# Autodesk Inventor assembly: Weapon Assembly
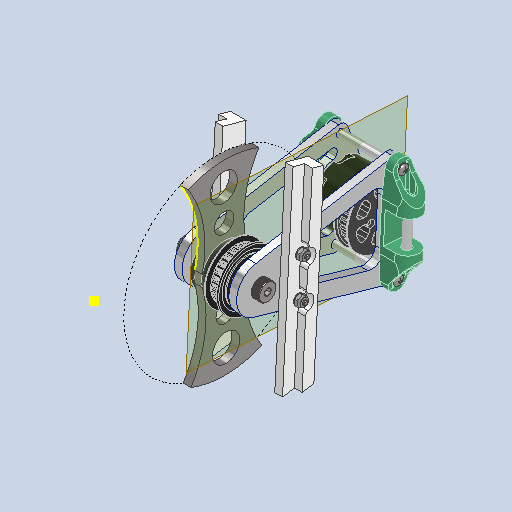
[picture p0: Inventor's stored thumbnail of the model, 512x512]
Saved by Autodesk Inventor 2023.1 (Build 271208000, 208)
## iProperties
Created: 2022-05-21
Part Number: Weapon Assembly
Document SubType Name: Assembly
Designer: Nathan Cai
Mass: 747.016 g
Surface Area: 1345.14 cm^2
Volume: 239.025 cm^3
Density: 3.12526 g/cm^3
Author: Nathan Cai
## Documents named in this file (15)
- C:\Users\Nathan Cai\Documents\Inventor\0.3rd Lawette - V3.5\Vertical Weapon Assembly (Type A - Low Power)\Weapon Assembly (Vert A - Low Power).iam
- C:\Users\Nathan Cai\Documents\Inventor\0.3rd Lawette - V3.5\Vertical Weapon Assembly (Type A)\90807A139_Same-Size Thread Alloy Steel Shoulder Screw.ipt
- C:\Users\Nathan Cai\Documents\Inventor\0.3rd Lawette - V3.5\Vertical Weapon Assembly (Type A)\90630A121_High-Strength Steel Nylon-Insert Locknut.ipt
- C:\Users\Nathan Cai\Documents\Inventor\0.3rd Lawette - V3.5\Vertical Weapon Assembly (Type A)\Frame (Clear Side).ipt
- C:\Users\Nathan Cai\Documents\Inventor\0.3rd Lawette - V3.5\Standoff 1.5in.ipt
- C:\Users\Nathan Cai\Documents\Inventor\0.3rd Lawette - V3.5\Vertical Weapon Assembly (Type A)\Legs.ipt
- C:\Users\Nathan Cai\Documents\Inventor\Content Center Files\R2023\en-US\ANSI B18.6.3(27)\ANSI B18.6.3 - 6-32 UNC - 0.75(11).ipt
- C:\Users\Nathan Cai\Documents\Inventor\Content Center Files\R2023\en-US\SAE J773b\SAE J773b - No. 6. SAE Type L. narrow.ipt
- C:\Users\Nathan Cai\Documents\Inventor\Content Center Files\R2023\en-US\IFI 100 107(2)\IFI 100_107 - No. 6 - 32 Metal Type.ipt
- C:\Users\Nathan Cai\Documents\Inventor\0.3rd Lawette - V3.5\Vertical Weapon Assembly (Type A)\Frame (Motor Side).ipt
- C:\Users\Nathan Cai\Documents\Inventor\0.3rd Lawette - V3.5\Vertical Weapon Assembly (Type A)\Legs_MIR.ipt
- C:\Users\Nathan Cai\Documents\Inventor\0.3rd Lawette - V3.5\Bracket.ipt
- C:\Users\Nathan Cai\Documents\Inventor\Content Center Files\R2023\en-US\ANSI B18.6.3(27)\ANSI B18.6.3 - 6-32 UNC - 0.625(11).ipt
- C:\Users\Nathan Cai\Documents\Inventor\0.3rd Lawette - V3.5\Vertical Weapon Assembly (Type A - Low Power)\Weapon (Weapon-Side Pulley).iam
- C:\Users\Nathan Cai\Documents\Inventor\0.3rd Lawette - V3.5\Vertical Weapon Assembly (Type A - Low Power)\Weapon (Motor-Side Pulley).iam
## Components (42 placed, 14 different names)
1. Weapon (Weapon-Side Pulley):2 [sub-assembly]
2. Weapon (Motor-Side Pulley):2 [sub-assembly]
3. 90807A139_Same-Size Thread Alloy Steel Shoulder Screw:1 — Mate:1, Mate:2, Mate:9, Mate:10
4. 90630A121_High-Strength Steel Nylon-Insert Locknut:1 — Mate:1, Mate:2
5. Frame (Motor Side):1 — Symmetry:1, Mate:146, Mate:147, Mate:148, Mate:170, Mate:194, Mate:195, Mate:196, Mate:197, Mate:198, Mate:200
6. Frame (Clear Side):1 — Mate:9, Mate:10, Mate:28, Mate:29, Mate:30, Mate:102, Symmetry:1, Mate:173, Mate:202, Mate:203, Mate:204, Mate:205, Mate:206, Mate:208
7. Legs:1 — Mate:28, Mate:29, Mate:30, Mate:207, Mate:209
8. Legs_MIR:1 — Mate:146, Mate:147, Mate:148, Mate:199, Mate:201
9. Bracket:1 — Mate:173, Mate:174, Mate:175, Mate:176, Flush:2, Mate:210, Mate:211, Mate:212, Mate:213, Mate:218, Mate:219, Mate:221, Mate:222
10. Bracket:2 — Mate:170, Mate:171, Mate:172, Mate:177, Flush:1, Mate:214, Mate:215, Mate:216, Mate:217, Mate:220, Mate:224
11. Standoff 1.5in:1 — Mate:102, Mate:171, Mate:174
12. Standoff 1.5in:2 — Mate:172, Mate:175
13. Standoff 1.5in:3 — Mate:176, Flush:2, Mate:223, Mate:225
14. Standoff 1.5in:4 — Mate:177, Flush:1
15. Cross Recessed Truss Head Machine Screw - Type I - Inch No. 6 - 32 - 5/8:8 — Insert:44
16. Conical Spring Washer SAE J773b (Inch) No. 6. SAE Type L. narrow:38 — Mate:224, Mate:225, Insert:44
17. Cross Recessed Truss Head Machine Screw - Type I - Inch No. 6 - 32 - 5/8:7 — Insert:43
18. Conical Spring Washer SAE J773b (Inch) No. 6. SAE Type L. narrow:37 — Mate:222, Mate:223, Insert:43
19. Cross Recessed Truss Head Machine Screw - Type I - Inch No. 6 - 32 - 5/8:6 — Insert:42
20. Conical Spring Washer SAE J773b (Inch) No. 6. SAE Type L. narrow:36 — Mate:220, Mate:221, Insert:42
21. Cross Recessed Truss Head Machine Screw - Type I - Inch No. 6 - 32 - 5/8:5 — Insert:41
22. Conical Spring Washer SAE J773b (Inch) No. 6. SAE Type L. narrow:35 — Mate:218, Mate:219, Insert:41
23. Cross Recessed Truss Head Machine Screw - Type I - Inch No. 6 - 32 - 3/4:27 — Insert:40
24. Conical Spring Washer SAE J773b (Inch) No. 6. SAE Type L. narrow:34 — Mate:216, Mate:217, Insert:40
25. Cross Recessed Truss Head Machine Screw - Type I - Inch No. 6 - 32 - 3/4:26 — Insert:39
26. Conical Spring Washer SAE J773b (Inch) No. 6. SAE Type L. narrow:33 — Mate:214, Mate:215, Insert:39
27. Cross Recessed Truss Head Machine Screw - Type I - Inch No. 6 - 32 - 3/4:25 — Insert:38
28. Conical Spring Washer SAE J773b (Inch) No. 6. SAE Type L. narrow:32 — Mate:212, Mate:213, Insert:38
29. Cross Recessed Truss Head Machine Screw - Type I - Inch No. 6 - 32 - 3/4:24 — Insert:37
30. Conical Spring Washer SAE J773b (Inch) No. 6. SAE Type L. narrow:31 — Mate:210, Mate:211, Insert:37
31. Prevailing Torque Type Hex Nut - Inch (IFI) No. 6 - 32 Metal Type:22 — Insert:36
32. Conical Spring Washer SAE J773b (Inch) No. 6. SAE Type L. narrow:30 — Mate:208, Mate:209, Insert:36
33. Cross Recessed Truss Head Machine Screw - Type I - Inch No. 6 - 32 - 3/4:23 — Mate:204, Mate:205
34. Prevailing Torque Type Hex Nut - Inch (IFI) No. 6 - 32 Metal Type:21 — Insert:35
35. Conical Spring Washer SAE J773b (Inch) No. 6. SAE Type L. narrow:29 — Mate:206, Mate:207, Insert:35
36. Cross Recessed Truss Head Machine Screw - Type I - Inch No. 6 - 32 - 3/4:22 — Mate:202, Mate:203
37. Prevailing Torque Type Hex Nut - Inch (IFI) No. 6 - 32 Metal Type:20 — Insert:34
38. Conical Spring Washer SAE J773b (Inch) No. 6. SAE Type L. narrow:28 — Mate:200, Mate:201, Insert:34
39. Cross Recessed Truss Head Machine Screw - Type I - Inch No. 6 - 32 - 3/4:21 — Mate:196, Mate:197
40. Prevailing Torque Type Hex Nut - Inch (IFI) No. 6 - 32 Metal Type:19 — Insert:33
41. Conical Spring Washer SAE J773b (Inch) No. 6. SAE Type L. narrow:27 — Mate:198, Mate:199, Insert:33
42. Cross Recessed Truss Head Machine Screw - Type I - Inch No. 6 - 32 - 3/4:20 — Mate:194, Mate:195
## Relationships (77: Mate 62, Insert 12, Flush 2, Symmetry 1)
- Mate:1: 90807A139_Same-Size Thread Alloy Steel Shoulder Screw:1 ↔ 90630A121_High-Strength Steel Nylon-Insert Locknut:1
- Mate:2 (50.8 mm): 90807A139_Same-Size Thread Alloy Steel Shoulder Screw:1 ↔ 90630A121_High-Strength Steel Nylon-Insert Locknut:1
- [Mate]: Weapon (Weapon-Side Pulley):2 ↔ 90807A139_Same-Size Thread Alloy Steel Shoulder Screw:1
- [Mate]: 90807A139_Same-Size Thread Alloy Steel Shoulder Screw:1 ↔ Frame (Motor Side):1
- Mate:9: 90807A139_Same-Size Thread Alloy Steel Shoulder Screw:1 ↔ Frame (Clear Side):1
- Mate:10: 90807A139_Same-Size Thread Alloy Steel Shoulder Screw:1 ↔ Frame (Clear Side):1
- [Mate]: Frame (Motor Side):1 ↔ Frame (Clear Side):1
- [Mate]: Frame (Motor Side):1 ↔ Standoff 1.5in:1
- [Mate]: Frame (Motor Side):1 ↔ Standoff 1.5in:2
- [Mate]: Frame (Motor Side):1 ↔ Standoff 1.5in:1
- [Mate]: Frame (Motor Side):1 ↔ Standoff 1.5in:2
- Mate:28: Frame (Clear Side):1 ↔ Legs:1
- Mate:29: Frame (Clear Side):1 ↔ Legs:1
- Mate:30: Frame (Clear Side):1 ↔ Legs:1
- Mate:102: Frame (Clear Side):1 ↔ Standoff 1.5in:1
- [Mate] (0.0254 mm): Weapon (Weapon-Side Pulley):2 ↔ Frame (Motor Side):1
- Symmetry:1: Frame (Motor Side):1 ↔ Frame (Clear Side):1
- Mate:146: Frame (Motor Side):1 ↔ Legs_MIR:1
- Mate:147: Frame (Motor Side):1 ↔ Legs_MIR:1
- Mate:148: Frame (Motor Side):1 ↔ Legs_MIR:1
- [Mate]: Weapon (Motor-Side Pulley):2 ↔ Frame (Motor Side):1
- [Mate]: Weapon (Motor-Side Pulley):2 ↔ Frame (Motor Side):1
- [Mate]: Weapon (Motor-Side Pulley):2 ↔ Frame (Motor Side):1
- Mate:170: Frame (Motor Side):1 ↔ Bracket:2
- Mate:171: Bracket:2 ↔ Standoff 1.5in:1
- Mate:172: Bracket:2 ↔ Standoff 1.5in:2
- Mate:173: Frame (Clear Side):1 ↔ Bracket:1
- Mate:174: Bracket:1 ↔ Standoff 1.5in:1
- Mate:175: Bracket:1 ↔ Standoff 1.5in:2
- Mate:176: Bracket:1 ↔ Standoff 1.5in:3
- Mate:177: Bracket:2 ↔ Standoff 1.5in:4
- Flush:1: Bracket:2 ↔ Standoff 1.5in:4
- Flush:2: Bracket:1 ↔ Standoff 1.5in:3
- Mate:194: Frame (Motor Side):1 ↔ Cross Recessed Truss Head Machine Screw - Type I - Inch No. 6 - 32 - 3/4:20
- Mate:195: Frame (Motor Side):1 ↔ Cross Recessed Truss Head Machine Screw - Type I - Inch No. 6 - 32 - 3/4:20
- Mate:196: Frame (Motor Side):1 ↔ Cross Recessed Truss Head Machine Screw - Type I - Inch No. 6 - 32 - 3/4:21
- Mate:197: Frame (Motor Side):1 ↔ Cross Recessed Truss Head Machine Screw - Type I - Inch No. 6 - 32 - 3/4:21
- Mate:198: Frame (Motor Side):1 ↔ Conical Spring Washer SAE J773b (Inch) No. 6. SAE Type L. narrow:27
- Mate:199: Legs_MIR:1 ↔ Conical Spring Washer SAE J773b (Inch) No. 6. SAE Type L. narrow:27
- Mate:200: Frame (Motor Side):1 ↔ Conical Spring Washer SAE J773b (Inch) No. 6. SAE Type L. narrow:28
- Mate:201: Legs_MIR:1 ↔ Conical Spring Washer SAE J773b (Inch) No. 6. SAE Type L. narrow:28
- Insert:33: Prevailing Torque Type Hex Nut - Inch (IFI) No. 6 - 32 Metal Type:19 ↔ Conical Spring Washer SAE J773b (Inch) No. 6. SAE Type L. narrow:27
- Insert:34: Prevailing Torque Type Hex Nut - Inch (IFI) No. 6 - 32 Metal Type:20 ↔ Conical Spring Washer SAE J773b (Inch) No. 6. SAE Type L. narrow:28
- Mate:202: Frame (Clear Side):1 ↔ Cross Recessed Truss Head Machine Screw - Type I - Inch No. 6 - 32 - 3/4:22
- Mate:203: Frame (Clear Side):1 ↔ Cross Recessed Truss Head Machine Screw - Type I - Inch No. 6 - 32 - 3/4:22
- Mate:204: Frame (Clear Side):1 ↔ Cross Recessed Truss Head Machine Screw - Type I - Inch No. 6 - 32 - 3/4:23
- Mate:205: Frame (Clear Side):1 ↔ Cross Recessed Truss Head Machine Screw - Type I - Inch No. 6 - 32 - 3/4:23
- Mate:206: Frame (Clear Side):1 ↔ Conical Spring Washer SAE J773b (Inch) No. 6. SAE Type L. narrow:29
- Mate:207: Legs:1 ↔ Conical Spring Washer SAE J773b (Inch) No. 6. SAE Type L. narrow:29
- Mate:208: Frame (Clear Side):1 ↔ Conical Spring Washer SAE J773b (Inch) No. 6. SAE Type L. narrow:30
- Mate:209: Legs:1 ↔ Conical Spring Washer SAE J773b (Inch) No. 6. SAE Type L. narrow:30
- Insert:35: Prevailing Torque Type Hex Nut - Inch (IFI) No. 6 - 32 Metal Type:21 ↔ Conical Spring Washer SAE J773b (Inch) No. 6. SAE Type L. narrow:29
- Insert:36: Prevailing Torque Type Hex Nut - Inch (IFI) No. 6 - 32 Metal Type:22 ↔ Conical Spring Washer SAE J773b (Inch) No. 6. SAE Type L. narrow:30
- Mate:210: Bracket:1 ↔ Conical Spring Washer SAE J773b (Inch) No. 6. SAE Type L. narrow:31
- Mate:211: Bracket:1 ↔ Conical Spring Washer SAE J773b (Inch) No. 6. SAE Type L. narrow:31
- Mate:212: Bracket:1 ↔ Conical Spring Washer SAE J773b (Inch) No. 6. SAE Type L. narrow:32
- Mate:213: Bracket:1 ↔ Conical Spring Washer SAE J773b (Inch) No. 6. SAE Type L. narrow:32
- Insert:37: Cross Recessed Truss Head Machine Screw - Type I - Inch No. 6 - 32 - 3/4:24 ↔ Conical Spring Washer SAE J773b (Inch) No. 6. SAE Type L. narrow:31
- Insert:38: Cross Recessed Truss Head Machine Screw - Type I - Inch No. 6 - 32 - 3/4:25 ↔ Conical Spring Washer SAE J773b (Inch) No. 6. SAE Type L. narrow:32
- Mate:214: Bracket:2 ↔ Conical Spring Washer SAE J773b (Inch) No. 6. SAE Type L. narrow:33
- Mate:215: Bracket:2 ↔ Conical Spring Washer SAE J773b (Inch) No. 6. SAE Type L. narrow:33
- Mate:216: Bracket:2 ↔ Conical Spring Washer SAE J773b (Inch) No. 6. SAE Type L. narrow:34
- Mate:217: Bracket:2 ↔ Conical Spring Washer SAE J773b (Inch) No. 6. SAE Type L. narrow:34
- Insert:39: Cross Recessed Truss Head Machine Screw - Type I - Inch No. 6 - 32 - 3/4:26 ↔ Conical Spring Washer SAE J773b (Inch) No. 6. SAE Type L. narrow:33
- Insert:40: Cross Recessed Truss Head Machine Screw - Type I - Inch No. 6 - 32 - 3/4:27 ↔ Conical Spring Washer SAE J773b (Inch) No. 6. SAE Type L. narrow:34
- Mate:218: Bracket:1 ↔ Conical Spring Washer SAE J773b (Inch) No. 6. SAE Type L. narrow:35
- Mate:219: Bracket:1 ↔ Conical Spring Washer SAE J773b (Inch) No. 6. SAE Type L. narrow:35
- Mate:220: Bracket:2 ↔ Conical Spring Washer SAE J773b (Inch) No. 6. SAE Type L. narrow:36
- Mate:221: Bracket:1 ↔ Conical Spring Washer SAE J773b (Inch) No. 6. SAE Type L. narrow:36
- Insert:41: Cross Recessed Truss Head Machine Screw - Type I - Inch No. 6 - 32 - 5/8:5 ↔ Conical Spring Washer SAE J773b (Inch) No. 6. SAE Type L. narrow:35
- Insert:42: Cross Recessed Truss Head Machine Screw - Type I - Inch No. 6 - 32 - 5/8:6 ↔ Conical Spring Washer SAE J773b (Inch) No. 6. SAE Type L. narrow:36
- Mate:222: Bracket:1 ↔ Conical Spring Washer SAE J773b (Inch) No. 6. SAE Type L. narrow:37
- Mate:223: Standoff 1.5in:3 ↔ Conical Spring Washer SAE J773b (Inch) No. 6. SAE Type L. narrow:37
- Mate:224: Bracket:2 ↔ Conical Spring Washer SAE J773b (Inch) No. 6. SAE Type L. narrow:38
- Mate:225: Standoff 1.5in:3 ↔ Conical Spring Washer SAE J773b (Inch) No. 6. SAE Type L. narrow:38
- Insert:43: Cross Recessed Truss Head Machine Screw - Type I - Inch No. 6 - 32 - 5/8:7 ↔ Conical Spring Washer SAE J773b (Inch) No. 6. SAE Type L. narrow:37
- Insert:44: Cross Recessed Truss Head Machine Screw - Type I - Inch No. 6 - 32 - 5/8:8 ↔ Conical Spring Washer SAE J773b (Inch) No. 6. SAE Type L. narrow:38
